# Autodesk Inventor assembly: Cup_Dispenser
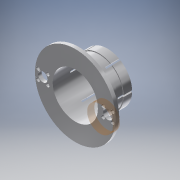
[picture p0: Inventor's stored thumbnail of the model, 180x180]
Saved by Autodesk Inventor 2016 (Build 200138000, 138)
## iProperties
Created: 2015-07-19
Part Number: Cup_Dispenser
Document SubType Name: Assembly
Designer: bastli
Author: bastli
## Documents named in this file (3)
- C:\Users\bastli\Documents\GitHub\BarBot\Conception\Mechanical\Cup_Dispenser_3\Cup_Dispenser.iam
- C:\Users\bastli\Documents\GitHub\BarBot\Conception\Mechanical\Cup_Dispenser_3\Fixture.ipt
- C:\Users\bastli\Documents\GitHub\BarBot\Conception\Mechanical\Cup_Dispenser_3\Transmission.ipt
## Components (2 placed, 2 different names)
1. Fixture:1 — Flush:1, Flush:2
2. Transmission:1 — Flush:1, Flush:2
## Relationships (2: Flush 2)
- Flush:1: Fixture:1 ↔ Transmission:1
- Flush:2 (1 mm): Fixture:1 ↔ Transmission:1
